# Autodesk Inventor assembly: 射出_腕
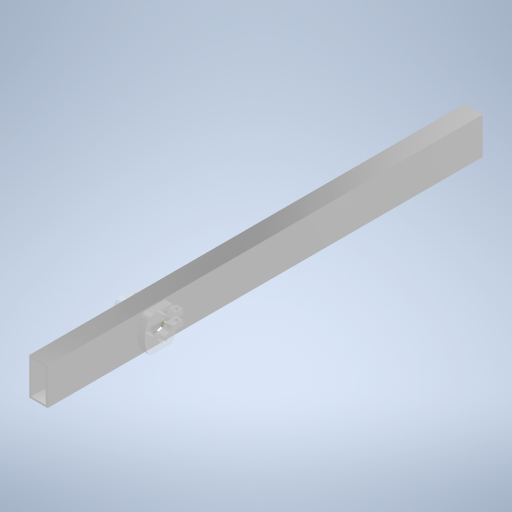
[picture p0: Inventor's stored thumbnail of the model, 512x512]
Saved by Autodesk Inventor 2023 (Build 270158000, 158)
## iProperties
Created: 2022-04-24
Part Number: 射出_腕
Document SubType Name: Assembly
Designer: yuta
Author: yuta
## Documents named in this file (3)
- C:\Users\yuta\Documents\NHK\射出_腕.iam
- C:\Users\yuta\Documents\NHK\射出_腕.ipt
- C:\Users\yuta\Documents\NHK\射出_腕固定.ipt
## Components (3 placed, 2 different names)
1. 射出_腕:1 — メイト:1, メイト:2, メイト:3, メイト:4
2. 射出_腕固定:1 — メイト:1, メイト:2
3. 射出_腕固定:2 — メイト:3, メイト:4
## Relationships (4: Mate 4)
- メイト:1 [Mate]: 射出_腕:1 ↔ 射出_腕固定:1
- メイト:2 [Mate]: 射出_腕:1 ↔ 射出_腕固定:1
- メイト:3 [Mate]: 射出_腕:1 ↔ 射出_腕固定:2
- メイト:4 [Mate]: 射出_腕:1 ↔ 射出_腕固定:2
